# Autodesk Inventor assembly: 組合1
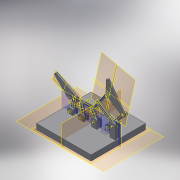
[picture p0: Inventor's stored thumbnail of the model, 180x180]
Saved by Autodesk Inventor 2017 (Build 210142000, 142)
## iProperties
Part Number: 組合1
Material: 一般
Document SubType Name: Assembly
Designer: 吳宜賢
Author: 吳宜賢
## Documents named in this file (13)
- C:\Users\吳宜賢\Desktop\組合1.iam
- C:\Users\吳宜賢\Desktop\零件1.ipt
- C:\Users\吳宜賢\Desktop\零件3.ipt
- C:\Users\吳宜賢\Desktop\零件4.ipt
- C:\Users\吳宜賢\Desktop\零件2.ipt
- C:\Users\吳宜賢\Desktop\零件5.ipt
- C:\Users\吳宜賢\Desktop\零件6.ipt
- C:\Users\吳宜賢\Desktop\零件7.ipt
- C:\Users\吳宜賢\Desktop\零件8.ipt
- C:\Users\吳宜賢\Desktop\零件9.ipt
- C:\Users\吳宜賢\Desktop\零件10.ipt
- C:\Users\吳宜賢\Desktop\零件11.ipt
- C:\Users\吳宜賢\Desktop\零件12.ipt
## Components (22 placed, 12 different names)
1. 零件1:1 — 貼合:1, 齊平:1, 貼合:2, 貼合:3, 貼合:8, 貼合:10, 貼合:11, 貼合:12, 貼合:19, 貼合:20, 貼合:24, 貼合:25, 貼合:27, 貼合:28, 貼合:29, 貼合:31, 貼合:33
2. 零件3:1 — 貼合:2, 貼合:3, 貼合:4, 貼合:5, 貼合:34, 齊平:2
3. 零件4:1 — 貼合:6, 貼合:7, 貼合:9, 貼合:13, 貼合:14
4. 零件2:1 — 貼合:4, 貼合:5, 貼合:6, 貼合:7, 貼合:35, 齊平:3
5. 零件5:1 — 貼合:8, 貼合:9, 貼合:10, 貼合:39
6. 零件6:1 — 貼合:11, 貼合:12, 貼合:13, 貼合:15, 貼合:32
7. 零件7:1 — 貼合:14, 貼合:15, 貼合:21, 貼合:22, 貼合:23, 貼合:37, 齊平:5
8. 零件8:1 — 貼合:24, 貼合:25, 貼合:26
9. 零件9:1 — 貼合:19, 貼合:20, 貼合:21, 貼合:36, 齊平:4
10. 零件10:1 — 貼合:22, 貼合:23, 貼合:26, 貼合:38, 齊平:6
11. 零件11:2 — 貼合:32
12. 零件11:5 — 貼合:27
13. 零件11:6 — 貼合:31
14. 零件11:8 — 貼合:29
15. 零件11:9 — 貼合:28
16. 零件11:10 — 貼合:33
17. 零件12:5 — 貼合:38, 齊平:6
18. 零件12:6 — 貼合:35, 齊平:3
19. 零件12:7 — 貼合:34, 齊平:2
20. 零件12:8 — 貼合:36, 齊平:4
21. 零件12:9 — 貼合:37, 齊平:5
22. 零件11:11 — 貼合:39
## Relationships (41: Mate 35, Flush 6)
- 貼合:1 [Mate]: 零件1:1
- 齊平:1 [Flush]: 零件1:1
- 貼合:2 [Mate]: 零件1:1 ↔ 零件3:1
- 貼合:3 [Mate]: 零件1:1 ↔ 零件3:1
- 貼合:4 [Mate]: 零件3:1 ↔ 零件2:1
- 貼合:5 [Mate]: 零件3:1 ↔ 零件2:1
- 貼合:6 [Mate]: 零件4:1 ↔ 零件2:1
- 貼合:7 [Mate]: 零件4:1 ↔ 零件2:1
- 貼合:8 [Mate]: 零件1:1 ↔ 零件5:1
- 貼合:9 [Mate]: 零件4:1 ↔ 零件5:1
- 貼合:10 [Mate]: 零件1:1 ↔ 零件5:1
- 貼合:11 [Mate]: 零件1:1 ↔ 零件6:1
- 貼合:12 [Mate]: 零件1:1 ↔ 零件6:1
- 貼合:13 [Mate]: 零件4:1 ↔ 零件6:1
- 貼合:14 [Mate]: 零件4:1 ↔ 零件7:1
- 貼合:15 [Mate]: 零件6:1 ↔ 零件7:1
- 貼合:19 [Mate]: 零件1:1 ↔ 零件9:1
- 貼合:20 [Mate]: 零件1:1 ↔ 零件9:1
- 貼合:21 [Mate]: 零件7:1 ↔ 零件9:1
- 貼合:22 [Mate]: 零件7:1 ↔ 零件10:1
- 貼合:23 [Mate]: 零件7:1 ↔ 零件10:1
- 貼合:24 [Mate]: 零件1:1 ↔ 零件8:1
- 貼合:25 [Mate]: 零件1:1 ↔ 零件8:1
- 貼合:26 [Mate]: 零件8:1 ↔ 零件10:1
- 貼合:27 [Mate]: 零件1:1 ↔ 零件11:5
- 貼合:28 [Mate]: 零件1:1 ↔ 零件11:9
- 貼合:29 [Mate]: 零件1:1 ↔ 零件11:8
- 貼合:31 [Mate]: 零件1:1 ↔ 零件11:6
- 貼合:32 [Mate]: 零件6:1 ↔ 零件11:2
- 貼合:33 [Mate]: 零件1:1 ↔ 零件11:10
- 貼合:34 [Mate]: 零件3:1 ↔ 零件12:7
- 齊平:2 [Flush]: 零件3:1 ↔ 零件12:7
- 貼合:35 [Mate]: 零件2:1 ↔ 零件12:6
- 齊平:3 [Flush]: 零件2:1 ↔ 零件12:6
- 貼合:36 [Mate]: 零件9:1 ↔ 零件12:8
- 齊平:4 [Flush]: 零件9:1 ↔ 零件12:8
- 貼合:37 [Mate]: 零件7:1 ↔ 零件12:9
- 齊平:5 [Flush]: 零件7:1 ↔ 零件12:9
- 貼合:38 [Mate]: 零件10:1 ↔ 零件12:5
- 齊平:6 [Flush]: 零件10:1 ↔ 零件12:5
- 貼合:39 [Mate]: 零件5:1 ↔ 零件11:11
